# Autodesk Inventor assembly: _VK_Seitenzentrier-Station
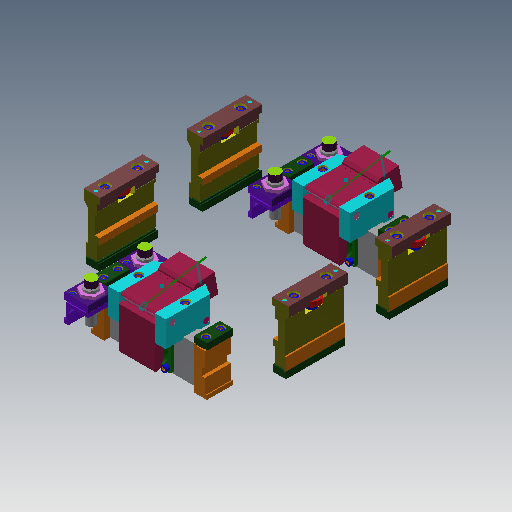
[picture p0: Inventor's stored thumbnail of the model, 512x512]
Saved by Autodesk Inventor 2019 (Build 230136000, 136)
## iProperties
Created: 2023-11-18
Part Number: _VK_Seitenzentrier-Station
Material: Generisch
Document SubType Name: Assembly
Designer: RP
Author: RP
## Documents named in this file (3)
- C:\Users\RP\Documents\Inventor\Projekt_Angelspule\_Verkettung\_VK_Seitenzentrier-Station.iam
- C:\Users\RP\Documents\Inventor\Projekt_Angelspule\_Verkettung\__VK_Stopper_Vor-Stopper_Einheit.iam
- C:\Users\RP\Documents\Inventor\Projekt_Angelspule\_Verkettung\__VK_Seitenzentrierung.ipt
## Components (5 placed, 2 different names)
1. __VK_Stopper_Vor-Stopper_Einheit:1 [sub-assembly]
2. __VK_Seitenzentrierung:1 — Fluchtend:30, Fluchtend:31, Fluchtend:35, Passend:6, Fluchtend:38
3. __VK_Seitenzentrierung:2 — Fluchtend:29, Fluchtend:30, Fluchtend:32, Fluchtend:34, Passend:7, Fluchtend:39
4. __VK_Seitenzentrierung:3 — Fluchtend:28, Fluchtend:29, Fluchtend:32, Passend:4, Fluchtend:36, Fluchtend:40
5. __VK_Seitenzentrierung:4 — Fluchtend:28, Fluchtend:31, Passend:5, Fluchtend:37, Fluchtend:41
## Relationships (17: Flush 13, Mate 4)
- Fluchtend:28 [Flush]: __VK_Seitenzentrierung:3 ↔ __VK_Seitenzentrierung:4
- Fluchtend:29 [Flush]: __VK_Seitenzentrierung:2 ↔ __VK_Seitenzentrierung:3
- Fluchtend:30 [Flush]: __VK_Seitenzentrierung:1 ↔ __VK_Seitenzentrierung:2
- Fluchtend:31 [Flush]: __VK_Seitenzentrierung:1 ↔ __VK_Seitenzentrierung:4
- Fluchtend:32 [Flush]: __VK_Seitenzentrierung:2 ↔ __VK_Seitenzentrierung:3
- Passend:4 [Mate] (127.25 mm): __VK_Seitenzentrierung:3
- Passend:5 [Mate] (127.25 mm): __VK_Seitenzentrierung:4
- Fluchtend:34 [Flush] (-127.25 mm): __VK_Seitenzentrierung:2
- Fluchtend:35 [Flush] (127.25 mm): __VK_Seitenzentrierung:1
- Fluchtend:36 [Flush] (-70 mm): __VK_Seitenzentrierung:3
- Passend:6 [Mate] (70 mm): __VK_Seitenzentrierung:1
- Fluchtend:37 [Flush] (-70 mm): __VK_Seitenzentrierung:4
- Passend:7 [Mate] (-70 mm): __VK_Seitenzentrierung:2
- Fluchtend:38 [Flush] (-10.415 mm): __VK_Seitenzentrierung:1
- Fluchtend:39 [Flush] (10.415 mm): __VK_Seitenzentrierung:2
- Fluchtend:40 [Flush] (10.415 mm): __VK_Seitenzentrierung:3
- Fluchtend:41 [Flush] (-10.415 mm): __VK_Seitenzentrierung:4
